# Autodesk Inventor assembly: mventosa+t
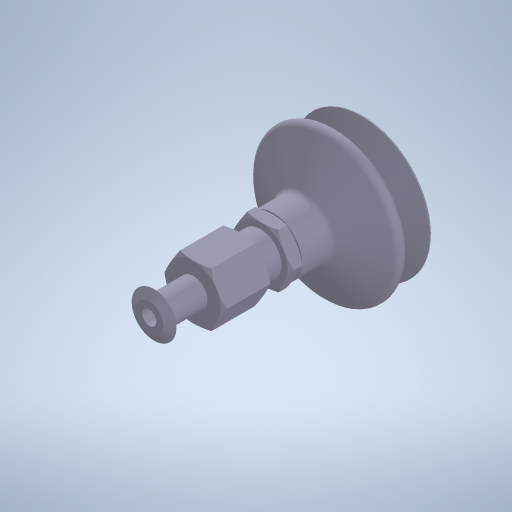
[picture p0: Inventor's stored thumbnail of the model, 512x512]
Saved by Autodesk Inventor 2023 (Build 270158000, 158)
## iProperties
Created: 2022-11-08
Part Number: mventosa+t
Document SubType Name: Assembly
Designer: Daniel
Author: Daniel
## Documents named in this file (4)
- D:\Documents\Universidad\Robotica\mventosa+t.iam
- D:\Documents\Universidad\Robotica\10_01_06_00874.ipt
- D:\Documents\Universidad\Robotica\10_01_06_01065.ipt
- D:\Documents\Universidad\Robotica\10_01_06_01066.ipt
## Components (3 placed, 3 different names)
1. 10_01_06_00874:1 — Cilíndrica:1, De rotación:1
2. 10_01_06_01065:1 — Cilíndrica:1, De rotación:1, Cilíndrica:2, De rotación:2
3. 10_01_06_01066:1 — Cilíndrica:2, De rotación:2
## Relationships (4: CylindricalJoint 2, RevoluteJoint 2)
- Cilíndrica:1 [CylindricalJoint]: 10_01_06_00874:1 ↔ 10_01_06_01065:1
- De rotación:1 [RevoluteJoint]: 10_01_06_00874:1 ↔ 10_01_06_01065:1
- Cilíndrica:2 [CylindricalJoint]: 10_01_06_01065:1 ↔ 10_01_06_01066:1
- De rotación:2 [RevoluteJoint] (6 mm): 10_01_06_01065:1 ↔ 10_01_06_01066:1
